# Autodesk Inventor assembly: sub_assy_robot_arm_link2
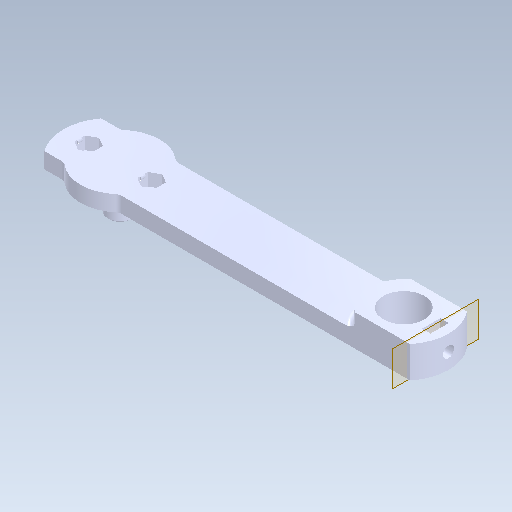
[picture p0: Inventor's stored thumbnail of the model, 512x512]
Saved by Autodesk Inventor 2021 (Build 250183000, 183)
## iProperties
Created: 2021-01-13
Part Number: sub_assy_robot_arm_link2
Document SubType Name: Assembly
Designer: Sam
Sending System: SolidWorks 2020
Last Author: Ben
Last Saved: 2021-01-14
Author: Sam
## Documents named in this file (3)
- D:\OneDrive\MSc Robotics\GIC\RobotKinematics-Remote\3D CAD\Autodesk\15012021\sub_assy_robot_arm_link2.iam
- D:\OneDrive\MSc Robotics\GIC\RobotKinematics-Remote\3D CAD\Autodesk\15012021\robot_arm_link_bearing_insert_mk1.ipt
- D:\OneDrive\MSc Robotics\GIC\RobotKinematics-Remote\3D CAD\Autodesk\15012021\arm_2_v1.ipt
## Components (2 placed, 2 different names)
1. arm_2_v1:1 — Mate:1, Mate:2, Mate:3
2. robot_arm_link_bearing_insert_mk1:1 — Mate:1, Mate:2, Mate:3
## Relationships (3: Mate 3)
- Mate:1: arm_2_v1:1 ↔ robot_arm_link_bearing_insert_mk1:1
- Mate:2: arm_2_v1:1 ↔ robot_arm_link_bearing_insert_mk1:1
- Mate:3: arm_2_v1:1 ↔ robot_arm_link_bearing_insert_mk1:1
